# Autodesk Inventor assembly: Tensionador_Cabos
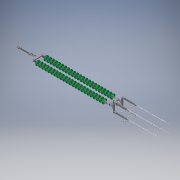
[picture p0: Inventor's stored thumbnail of the model, 180x180]
Saved by Autodesk Inventor 2018 (Build 220112000, 112)
## iProperties
Created: 2021-04-28
Part Number: Tensionador_Cabos
Document SubType Name: Assembly
Designer: l01767
Author: l01767
## Documents named in this file (15)
- F:\Projetos\TAESA\Modelo 3D - Tensionadores e Suspensão\Tensionador\Tensionador-5-Cabos.iam
- F:\Projetos\TAESA\Modelo 3D - Tensionadores e Suspensão\Tensionador\gpghmb32.iam
- F:\Projetos\TAESA\Modelo 3D - Tensionadores e Suspensão\Tensionador\Link_Principal.ipt
- F:\Projetos\TAESA\Modelo 3D - Tensionadores e Suspensão\Tensionador\Espacador_Delta.ipt
- F:\Projetos\TAESA\Modelo 3D - Tensionadores e Suspensão\Tensionador\Clevis-Bola_Curto.ipt
- F:\Projetos\TAESA\Modelo 3D - Tensionadores e Suspensão\Tensionador\Bolted Connection1.iam
- F:\Projetos\TAESA\Modelo 3D - Tensionadores e Suspensão\Tensionador\U300B.iam
- F:\Projetos\TAESA\Modelo 3D - Tensionadores e Suspensão\Tensionador\Clevis-Socket.iam
- F:\Projetos\TAESA\Modelo 3D - Tensionadores e Suspensão\Tensionador\Balancim_Duplicador.ipt
- F:\Projetos\TAESA\Modelo 3D - Tensionadores e Suspensão\Tensionador\gpghmb22.iam
- F:\Projetos\TAESA\Modelo 3D - Tensionadores e Suspensão\Tensionador\Espacador_Delta_Secundario.ipt
- F:\Projetos\TAESA\Modelo 3D - Tensionadores e Suspensão\Tensionador\OPGW Tension set.iam
- F:\Projetos\TAESA\Modelo 3D - Tensionadores e Suspensão\Tensionador\Link_Tensionador.ipt
- F:\Projetos\TAESA\Modelo 3D - Tensionadores e Suspensão\Tensionador\Bolted Connection3.iam
- F:\Projetos\TAESA\Modelo 3D - Tensionadores e Suspensão\Tensionador\Bolted Connection4.iam
## Components (83 placed, 12 different names)
1. gpghmb32:1 [sub-assembly] — Mate:1, Mate:2, Flush:1, Mate:3, Mate:4, Mate:6
2. gpghmb32:2 [sub-assembly] — Mate:5, Mate:7, Flush:2, Flush:11, Flush:10, Tangent:1
3. Link_Principal:1 — Mate:1, Mate:4, Mate:5, Mate:6, Mate:7, Flush:2
4. gpghmb32:3 [sub-assembly] — Flush:11, Flush:10, Tangent:1, Mate:8, Mate:9, Mate:10
5. Espacador_Delta:1 — Mate:8, Mate:9, Mate:10, Mate:11, Angle:1, Mate:12
6. Clevis-Socket:1 [sub-assembly] — Mate:23, Mate:24, Mate:30
7. Clevis-Socket:3 [sub-assembly] — Mate:27, Mate:28, Mate:29
8. Balancim_Duplicador:1 — Mate:29, Mate:30, Mate:32, Mate:33, Flush:12, Mate:34, Mate:35, Mate:36, Mate:37, Mate:38, Angle:10, Angle:11
9. gpghmb32:4 [sub-assembly] — Mate:32, Mate:33, Flush:12, Flush:13, Flush:14, Tangent:2
10. gpghmb32:5 [sub-assembly] — Flush:13, Flush:14, Tangent:2, Mate:45
11. gpghmb22:1 [sub-assembly] — Mate:34, Mate:35, Flush:15, Tangent:3
12. gpghmb22:2 [sub-assembly] — Mate:36, Flush:15, Tangent:3, Mate:41, Flush:16, Flush:17
13. gpghmb22:3 [sub-assembly] — Mate:37, Mate:38, Mate:39, Mate:40, Tangent:4
14. gpghmb22:4 [sub-assembly] — Mate:39, Mate:40, Tangent:4, Mate:42, Mate:43, Mate:44
15. Espacador_Delta_Secundario:1 — Mate:41, Flush:16, Flush:17
16. Espacador_Delta_Secundario:2 — Mate:42, Mate:43, Mate:44, Mate:46, Mate:47
17. OPGW Tension set:1 [sub-assembly] — Mate:45, Angle:10
18. Clevis-Bola_Curto:1 — Mate:11, Angle:1, Mate:12, Mate:13, Mate:14, Mate:15, Mate:16, Angle:2
19. Bolted Connection:1 [sub-assembly] — Mate:13, Mate:14
20. Clevis-Bola_Curto:2
21. Bolted Connection:2 [sub-assembly]
22. Link_Tensionador:1 — Mate:46, Mate:47, Angle:11, Mate:48, Mate:49, Mate:50, Angle:12, Mate:51, Mate:52, Mate:53
23. Bolted Connection:4 [sub-assembly] — Mate:48, Mate:49
24. OPGW Tension set:2 [sub-assembly] — Mate:50, Angle:12, Mate:51
25. Bolted Connection:5 [sub-assembly] — Mate:52, Mate:53
26. Link_Tensionador:2
27. Bolted Connection:6 [sub-assembly]
28. OPGW Tension set:3 [sub-assembly]
29. Bolted Connection:7 [sub-assembly]
30. Link_Tensionador:3
31. Bolted Connection:8 [sub-assembly]
32. OPGW Tension set:4 [sub-assembly]
33. Bolted Connection:9 [sub-assembly]
34. Link_Tensionador:4
35. Bolted Connection:10 [sub-assembly]
36. OPGW Tension set:5 [sub-assembly]
37. Bolted Connection:11 [sub-assembly]
38. U300B:1 [sub-assembly] — Mate:15, Mate:16, Angle:2
39. U300B:2 [sub-assembly]
40. U300B:3 [sub-assembly]
41. U300B:4 [sub-assembly]
42. U300B:5 [sub-assembly]
43. U300B:6 [sub-assembly]
44. U300B:7 [sub-assembly]
45. U300B:8 [sub-assembly]
46. U300B:9 [sub-assembly]
47. U300B:10 [sub-assembly]
48. U300B:11 [sub-assembly]
49. U300B:12 [sub-assembly]
50. U300B:13 [sub-assembly]
51. U300B:14 [sub-assembly]
52. U300B:15 [sub-assembly]
53. U300B:16 [sub-assembly]
54. U300B:17 [sub-assembly]
55. U300B:18 [sub-assembly]
56. U300B:19 [sub-assembly]
57. U300B:20 [sub-assembly]
58. U300B:21 [sub-assembly]
59. U300B:22 [sub-assembly]
60. U300B:23 [sub-assembly] — Mate:23, Mate:24
61. U300B:24 [sub-assembly]
62. U300B:25 [sub-assembly]
63. U300B:26 [sub-assembly]
64. U300B:27 [sub-assembly]
65. U300B:28 [sub-assembly]
66. U300B:29 [sub-assembly]
67. U300B:30 [sub-assembly]
68. U300B:31 [sub-assembly]
69. U300B:32 [sub-assembly]
70. U300B:33 [sub-assembly]
71. U300B:34 [sub-assembly]
72. U300B:35 [sub-assembly]
73. U300B:36 [sub-assembly]
74. U300B:37 [sub-assembly]
75. U300B:38 [sub-assembly]
76. U300B:39 [sub-assembly]
77. U300B:40 [sub-assembly]
78. U300B:41 [sub-assembly]
79. U300B:42 [sub-assembly]
80. U300B:43 [sub-assembly]
81. U300B:44 [sub-assembly]
82. U300B:45 [sub-assembly]
83. U300B:46 [sub-assembly] — Mate:27, Mate:28
## Component patterns: (2 elements, first: Clevis-Bola_Curto:1 + Bolted Connection:1), (4 elements, first: Link_Tensionador:1 + Bolted Connection:4 + OPGW Tension set:2 + Bolted Connection:5), (23 elements, first: U300B:1), Component Pattern 1:2 (23 elements)
## Relationships (63: Mate 44, Flush 10, Angle 5, Tangent 4)
- Mate:1: gpghmb32:1 ↔ Link_Principal:1
- Mate:2: gpghmb32:1
- Flush:1: gpghmb32:1
- Mate:3: gpghmb32:1
- Mate:4: gpghmb32:1 ↔ Link_Principal:1
- Mate:5: gpghmb32:2 ↔ Link_Principal:1
- Mate:6: gpghmb32:1 ↔ Link_Principal:1
- Mate:7: gpghmb32:2 ↔ Link_Principal:1
- Flush:2: gpghmb32:2 ↔ Link_Principal:1
- Flush:11: gpghmb32:2 ↔ gpghmb32:3
- Flush:10: gpghmb32:2 ↔ gpghmb32:3
- Tangent:1: gpghmb32:2 ↔ gpghmb32:3
- Mate:8: gpghmb32:3 ↔ Espacador_Delta:1
- Mate:9: gpghmb32:3 ↔ Espacador_Delta:1
- Mate:10: gpghmb32:3 ↔ Espacador_Delta:1
- Mate:11: Espacador_Delta:1 ↔ Clevis-Bola_Curto:1
- Angle:1 (180 deg): Espacador_Delta:1 ↔ Clevis-Bola_Curto:1
- Mate:12: Espacador_Delta:1 ↔ Clevis-Bola_Curto:1
- Mate:13: Clevis-Bola_Curto:1 ↔ Bolted Connection:1
- Mate:14: Clevis-Bola_Curto:1 ↔ Bolted Connection:1
- Mate:15: Clevis-Bola_Curto:1 ↔ U300B:1
- Mate:16 (5 mm): Clevis-Bola_Curto:1 ↔ U300B:1
- Angle:2 (0 deg): Clevis-Bola_Curto:1 ↔ U300B:1
- Mate:23: Clevis-Socket:1 ↔ U300B:23
- Mate:24 (15 mm): Clevis-Socket:1 ↔ U300B:23
- Mate:27: Clevis-Socket:3 ↔ U300B:46
- Mate:28 (15 mm): Clevis-Socket:3 ↔ U300B:46
- Mate:29: Clevis-Socket:3 ↔ Balancim_Duplicador:1
- Mate:30: Clevis-Socket:1 ↔ Balancim_Duplicador:1
- Mate:32: Balancim_Duplicador:1 ↔ gpghmb32:4
- Mate:33: Balancim_Duplicador:1 ↔ gpghmb32:4
- Flush:12: Balancim_Duplicador:1 ↔ gpghmb32:4
- Flush:13: gpghmb32:4 ↔ gpghmb32:5
- Flush:14: gpghmb32:4 ↔ gpghmb32:5
- Tangent:2: gpghmb32:4 ↔ gpghmb32:5
- Mate:34: Balancim_Duplicador:1 ↔ gpghmb22:1
- Mate:35: Balancim_Duplicador:1 ↔ gpghmb22:1
- Mate:36: Balancim_Duplicador:1 ↔ gpghmb22:2
- Flush:15: gpghmb22:1 ↔ gpghmb22:2
- Tangent:3: gpghmb22:1 ↔ gpghmb22:2
- Mate:37: Balancim_Duplicador:1 ↔ gpghmb22:3
- Mate:38: Balancim_Duplicador:1 ↔ gpghmb22:3
- Mate:39: gpghmb22:3 ↔ gpghmb22:4
- Mate:40: gpghmb22:3 ↔ gpghmb22:4
- Tangent:4: gpghmb22:3 ↔ gpghmb22:4
- Mate:41: gpghmb22:2 ↔ Espacador_Delta_Secundario:1
- Mate:42: gpghmb22:4 ↔ Espacador_Delta_Secundario:2
- Mate:43: gpghmb22:4 ↔ Espacador_Delta_Secundario:2
- Mate:44: gpghmb22:4 ↔ Espacador_Delta_Secundario:2
- Flush:16: gpghmb22:2 ↔ Espacador_Delta_Secundario:1
- Flush:17: gpghmb22:2 ↔ Espacador_Delta_Secundario:1
- Mate:45: gpghmb32:5 ↔ OPGW Tension set:1
- Angle:10 (0 deg): Balancim_Duplicador:1 ↔ OPGW Tension set:1
- Mate:46: Espacador_Delta_Secundario:2 ↔ Link_Tensionador:1
- Mate:47: Espacador_Delta_Secundario:2 ↔ Link_Tensionador:1
- Angle:11 (0 deg): Balancim_Duplicador:1 ↔ Link_Tensionador:1
- Mate:48: Link_Tensionador:1 ↔ Bolted Connection:4
- Mate:49: Link_Tensionador:1 ↔ Bolted Connection:4
- Mate:50: Link_Tensionador:1 ↔ OPGW Tension set:2
- Angle:12 (0 deg): Link_Tensionador:1 ↔ OPGW Tension set:2
- Mate:51 (2.5 mm): Link_Tensionador:1 ↔ OPGW Tension set:2
- Mate:52: Link_Tensionador:1 ↔ Bolted Connection:5
- Mate:53: Link_Tensionador:1 ↔ Bolted Connection:5
